# Autodesk Inventor assembly: Intake V3
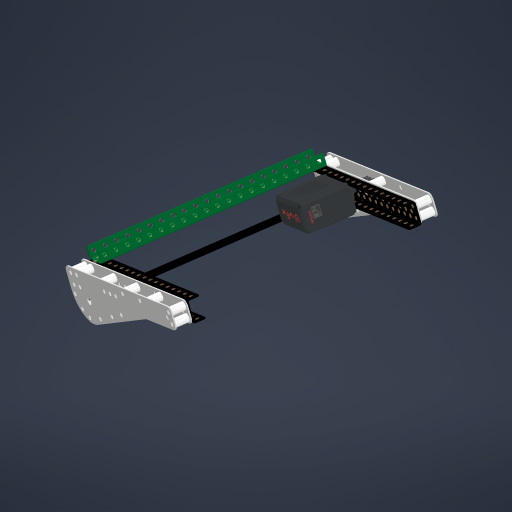
[picture p0: Inventor's stored thumbnail of the model, 512x512]
Saved by Autodesk Inventor 2023.4 (Build 274418000, 418)
## iProperties
Created: 2023-12-16
Part Number: Intake V3
Document SubType Name: Assembly
Designer: diego
Author: diego
## Documents named in this file (17)
- C:\Users\Meer\OneDrive\Documents\GitHub\2024-599Z\Cad\NEW Intake\plan x intake.iam
- C:\Users\Meer\OneDrive\Documents\GitHub\2024-599Z\Cad\Library\VEX-CAD-Inventor-1.4.0\Structure\C Channel\Aluminum 1x2x1\Alu C 1x2x1x17.ipt
- C:\Users\Meer\OneDrive\Documents\GitHub\2024-599Z\Cad\Library\VEX-CAD-Inventor-1.4.0\Motion\Shaft HS\HS Spacer\HSpacer .0625.ipt
- C:\Users\Meer\OneDrive\Documents\GitHub\2024-599Z\Cad\Library\VEX-CAD-Inventor-1.4.0\Motion\Shaft HS\Shaft HS\Shaft HS 11.0 in.ipt
- C:\Users\Meer\OneDrive\Documents\GitHub\2024-599Z\Cad\Library\VEX-CAD-Inventor-1.4.0\Motion\Sprockets\6P Sprocket\6P 8T Sprocket, No Insert.iam
- C:\Users\Meer\OneDrive\Documents\GitHub\2024-599Z\Cad\Library\VEX-CAD-Inventor-1.4.0\Motion\Shaft HS\Low Profile HS Shaft Collar.ipt
- C:\Users\Meer\OneDrive\Documents\GitHub\2024-599Z\Cad\Library\VEX-CAD-Inventor-1.4.0\Motion\Spacers\Spacer Nylon .313 OD\NSpacer .313 OD x .500.ipt
- C:\Users\Meer\OneDrive\Documents\GitHub\2024-599Z\Cad\Library\VEX-CAD-Inventor-1.4.0\Motion\Spacers\Spacer Nylon .313 OD.ipt
- C:\Users\Meer\OneDrive\Documents\GitHub\2024-599Z\Cad\Library\VEX-CAD-Inventor-1.4.0\Motion\Spacers\Spacer Nylon .313 OD\NSpacer .313 OD x .125.ipt
- C:\Users\Meer\OneDrive\Documents\GitHub\2024-599Z\Cad\Library\VEX-CAD-Inventor-1.4.0\Motion\Sprockets\6P Sprocket.iam
- C:\Users\Meer\OneDrive\Documents\GitHub\2024-599Z\Cad\Library\VEX-CAD-Inventor-1.4.0\Motion\Shaft HS\HS Spacer.ipt
- C:\Users\Meer\OneDrive\Documents\GitHub\2024-599Z\Cad\Library\VEX-CAD-Inventor-1.4.0\Motion\Sprockets\6P Sprocket\6P 8T Sprocket, Square.iam
- C:\Users\Meer\OneDrive\Documents\GitHub\2024-599Z\Cad\Library\VEX-CAD-Inventor-1.4.0\Structure\C Channel\Aluminum 1x2x1\Alu C 1x2x1x20.ipt
- C:\Users\Meer\OneDrive\Documents\GitHub\2024-599Z\Cad\Library\VEX-CAD-Inventor-1.4.0\Motion\Shaft HS\Shaft HS.ipt
- C:\Users\Meer\OneDrive\Documents\GitHub\2024-599Z\Cad\NEW CNC Poly\intake poly x.ipt
- C:\Users\Meer\OneDrive\Documents\GitHub\2024-599Z\Cad\Library\VEX-CAD-Inventor-1.4.0\Electronics\Motors with Screws\SteelM-StarS.iam
- C:\Users\Meer\OneDrive\Documents\GitHub\2024-599Z\Cad\Library\VEX-CAD-Inventor-1.4.0\Electronics\Motors with Screws.iam
## Components (78 placed, 11 different names)
1. Shaft HS 11.0 in:1
2. Alu C 1x2x1x17:1 — Insert:138, Insert:139, Insert:146, Insert:147, Insert:208, Insert:209
3. Alu C 1x2x1x17:2 — Insert:136, Insert:137, Insert:205, Insert:206
4. 6P 8T Sprocket, No Insert:4 [sub-assembly] — Insert:24, Insert:39
5. HSpacer .0625:8 — Insert:24
6. HSpacer .0625:12 — Insert:39
7. NSpacer .313 OD x .500:1 — Insert:71, Insert:160
8. NSpacer .313 OD x .500:2 — Insert:65, Insert:161
9. NSpacer .313 OD x .500:4 — Insert:72, Insert:159
10. NSpacer .313 OD x .500:6 — Insert:63, Insert:150
11. NSpacer .313 OD x .500:8 — Insert:74, Insert:157
12. NSpacer .313 OD x .500:9 — Insert:62
13. NSpacer .313 OD x .500:10 — Insert:61
14. NSpacer .313 OD x .500:12 — Insert:67, Insert:154
15. NSpacer .313 OD x .500:13 — Insert:73, Insert:158
16. NSpacer .313 OD x .500:15 — Insert:69, Insert:156
17. NSpacer .313 OD x .125:19 — Insert:61
18. NSpacer .313 OD x .125:20 — Insert:63
19. NSpacer .313 OD x .125:21 — Insert:65
20. NSpacer .313 OD x .125:23 — Insert:62, Insert:201
21. NSpacer .313 OD x .125:24 — Insert:67
22. NSpacer .313 OD x .125:26 — Insert:69, Insert:200
23. NSpacer .313 OD x .125:27 — Insert:71
24. NSpacer .313 OD x .125:29 — Insert:72
25. NSpacer .313 OD x .125:30 — Insert:73
26. NSpacer .313 OD x .125:31 — Insert:74
27. NSpacer .313 OD x .500:34 — Insert:163
28. NSpacer .313 OD x .500:35 — Insert:162
29. NSpacer .313 OD x .500:37 — Insert:153
30. NSpacer .313 OD x .125:47
31. NSpacer .313 OD x .125:50
32. NSpacer .313 OD x .125:59
33. Low Profile HS Shaft Collar:4
34. HSpacer .0625:14 — Insert:135
35. HSpacer .0625:15 — Insert:134, Insert:210
36. 6P 8T Sprocket, Square:6 [sub-assembly] — Insert:134, Insert:135
37. Alu C 1x2x1x20:1 — Insert:136, Insert:137, Insert:138, Insert:139
38. intake poly x:1 — Insert:146, Insert:147, Insert:150, Insert:153, Insert:154, Insert:156, Insert:157, Insert:158, Insert:159, Insert:160, Insert:161, Insert:162, Insert:163, Insert:210
39. intake poly x:2 — Insert:202, Insert:203, Insert:204, Insert:205, Insert:206
40. NSpacer .313 OD x .500:65
41. NSpacer .313 OD x .500:66
42. NSpacer .313 OD x .500:67
43. NSpacer .313 OD x .500:68
44. NSpacer .313 OD x .500:69
45. NSpacer .313 OD x .500:70
46. NSpacer .313 OD x .500:71
47. NSpacer .313 OD x .500:72
48. NSpacer .313 OD x .500:73 — Insert:198
49. NSpacer .313 OD x .500:74 — Insert:199
50. NSpacer .313 OD x .500:75
51. NSpacer .313 OD x .500:76
52. NSpacer .313 OD x .500:77
53. NSpacer .313 OD x .500:78
54. NSpacer .313 OD x .500:79
55. NSpacer .313 OD x .125:80
56. NSpacer .313 OD x .125:81
57. NSpacer .313 OD x .125:82 — Insert:203
58. NSpacer .313 OD x .125:83
59. NSpacer .313 OD x .125:84
60. NSpacer .313 OD x .125:85
61. NSpacer .313 OD x .125:86 — Insert:204
62. NSpacer .313 OD x .125:87
63. NSpacer .313 OD x .125:88
64. NSpacer .313 OD x .125:89 — Insert:202
65. NSpacer .313 OD x .125:90
66. NSpacer .313 OD x .125:91
67. NSpacer .313 OD x .125:92
68. NSpacer .313 OD x .125:93
69. NSpacer .313 OD x .125:94
70. NSpacer .313 OD x .500:95
71. NSpacer .313 OD x .500:96
72. NSpacer .313 OD x .500:97
73. NSpacer .313 OD x .125:98
74. NSpacer .313 OD x .125:99
75. NSpacer .313 OD x .125:100
76. intake poly x:3 — Insert:198, Insert:199
77. intake poly x:4 — Insert:200, Insert:201
78. SteelM-StarS:1 [sub-assembly] — Insert:208, Insert:209
## Relationships (80: Insert 80)
- Insert:24: 6P 8T Sprocket, No Insert:4 ↔ HSpacer .0625:8
- Insert:39: 6P 8T Sprocket, No Insert:4 ↔ HSpacer .0625:12
- Insert:61: NSpacer .313 OD x .500:10 ↔ NSpacer .313 OD x .125:19
- Insert:62: NSpacer .313 OD x .500:9 ↔ NSpacer .313 OD x .125:23
- Insert:63: NSpacer .313 OD x .500:6 ↔ NSpacer .313 OD x .125:20
- Insert:65: NSpacer .313 OD x .500:2 ↔ NSpacer .313 OD x .125:21
- Insert:67: NSpacer .313 OD x .500:12 ↔ NSpacer .313 OD x .125:24
- Insert:69: NSpacer .313 OD x .500:15 ↔ NSpacer .313 OD x .125:26
- Insert:71: NSpacer .313 OD x .500:1 ↔ NSpacer .313 OD x .125:27
- Insert:72: NSpacer .313 OD x .500:4 ↔ NSpacer .313 OD x .125:29
- Insert:73: NSpacer .313 OD x .500:13 ↔ NSpacer .313 OD x .125:30
- Insert:74: NSpacer .313 OD x .500:8 ↔ NSpacer .313 OD x .125:31
- [Insert]: NSpacer .313 OD x .500:34 ↔ NSpacer .313 OD x .125:47
- [Insert]: NSpacer .313 OD x .500:37 ↔ NSpacer .313 OD x .125:50
- [Insert]: NSpacer .313 OD x .500:35 ↔ NSpacer .313 OD x .125:59
- Insert:134: HSpacer .0625:15 ↔ 6P 8T Sprocket, Square:6
- Insert:135: HSpacer .0625:14 ↔ 6P 8T Sprocket, Square:6
- Insert:136: Alu C 1x2x1x17:2 ↔ Alu C 1x2x1x20:1
- Insert:137: Alu C 1x2x1x17:2 ↔ Alu C 1x2x1x20:1
- Insert:138: Alu C 1x2x1x17:1 ↔ Alu C 1x2x1x20:1
- Insert:139: Alu C 1x2x1x17:1 ↔ Alu C 1x2x1x20:1
- Insert:146: Alu C 1x2x1x17:1 ↔ intake poly x:1
- Insert:147: Alu C 1x2x1x17:1 ↔ intake poly x:1
- Insert:150: NSpacer .313 OD x .500:6 ↔ intake poly x:1
- Insert:153: NSpacer .313 OD x .500:37 ↔ intake poly x:1
- Insert:154: NSpacer .313 OD x .500:12 ↔ intake poly x:1
- Insert:156: NSpacer .313 OD x .500:15 ↔ intake poly x:1
- Insert:157: NSpacer .313 OD x .500:8 ↔ intake poly x:1
- Insert:158: NSpacer .313 OD x .500:13 ↔ intake poly x:1
- Insert:159: NSpacer .313 OD x .500:4 ↔ intake poly x:1
- Insert:160: NSpacer .313 OD x .500:1 ↔ intake poly x:1
- Insert:161: NSpacer .313 OD x .500:2 ↔ intake poly x:1
- Insert:162: NSpacer .313 OD x .500:35 ↔ intake poly x:1
- Insert:163: NSpacer .313 OD x .500:34 ↔ intake poly x:1
- [Insert]: NSpacer .313 OD x .500:67 ↔ NSpacer .313 OD x .125:80
- [Insert]: NSpacer .313 OD x .500:71 ↔ NSpacer .313 OD x .125:81
- [Insert]: NSpacer .313 OD x .500:74 ↔ NSpacer .313 OD x .125:82
- [Insert]: NSpacer .313 OD x .500:73 ↔ NSpacer .313 OD x .125:86
- [Insert]: NSpacer .313 OD x .500:70 ↔ NSpacer .313 OD x .125:83
- [Insert]: NSpacer .313 OD x .500:75 ↔ NSpacer .313 OD x .125:85
- [Insert]: NSpacer .313 OD x .500:66 ↔ NSpacer .313 OD x .125:84
- [Insert]: NSpacer .313 OD x .500:69 ↔ NSpacer .313 OD x .125:88
- [Insert]: NSpacer .313 OD x .500:76 ↔ NSpacer .313 OD x .125:87
- [Insert]: NSpacer .313 OD x .500:78 ↔ NSpacer .313 OD x .125:91
- [Insert]: NSpacer .313 OD x .500:79 ↔ NSpacer .313 OD x .125:89
- [Insert]: NSpacer .313 OD x .500:65 ↔ NSpacer .313 OD x .125:90
- [Insert]: NSpacer .313 OD x .500:68 ↔ NSpacer .313 OD x .125:92
- [Insert]: NSpacer .313 OD x .500:77 ↔ NSpacer .313 OD x .125:93
- [Insert]: NSpacer .313 OD x .500:72 ↔ NSpacer .313 OD x .125:94
- [Insert]: NSpacer .313 OD x .500:95 ↔ NSpacer .313 OD x .125:98
- [Insert]: NSpacer .313 OD x .500:97 ↔ NSpacer .313 OD x .125:99
- [Insert]: NSpacer .313 OD x .500:96 ↔ NSpacer .313 OD x .125:100
- [Insert]: NSpacer .313 OD x .500:71 ↔ intake poly x:3
- [Insert]: NSpacer .313 OD x .500:67 ↔ intake poly x:3
- [Insert]: NSpacer .313 OD x .500:70 ↔ intake poly x:3
- [Insert]: NSpacer .313 OD x .500:75 ↔ intake poly x:3
- [Insert]: NSpacer .313 OD x .500:69 ↔ intake poly x:3
- [Insert]: NSpacer .313 OD x .500:97 ↔ intake poly x:3
- [Insert]: NSpacer .313 OD x .500:76 ↔ intake poly x:3
- [Insert]: NSpacer .313 OD x .500:78 ↔ intake poly x:3
- [Insert]: NSpacer .313 OD x .500:79 ↔ intake poly x:3
- [Insert]: NSpacer .313 OD x .500:72 ↔ intake poly x:3
- [Insert]: NSpacer .313 OD x .500:77 ↔ intake poly x:3
- [Insert]: NSpacer .313 OD x .500:68 ↔ intake poly x:3
- [Insert]: NSpacer .313 OD x .500:65 ↔ intake poly x:3
- [Insert]: NSpacer .313 OD x .500:66 ↔ intake poly x:3
- [Insert]: NSpacer .313 OD x .500:96 ↔ intake poly x:3
- [Insert]: NSpacer .313 OD x .500:95 ↔ intake poly x:3
- Insert:198: NSpacer .313 OD x .500:73 ↔ intake poly x:3
- Insert:199: NSpacer .313 OD x .500:74 ↔ intake poly x:3
- Insert:200: NSpacer .313 OD x .125:26 ↔ intake poly x:4
- Insert:201: NSpacer .313 OD x .125:23 ↔ intake poly x:4
- Insert:202: intake poly x:2 ↔ NSpacer .313 OD x .125:89
- Insert:203: intake poly x:2 ↔ NSpacer .313 OD x .125:82
- Insert:204: intake poly x:2 ↔ NSpacer .313 OD x .125:86
- Insert:205: Alu C 1x2x1x17:2 ↔ intake poly x:2
- Insert:206: Alu C 1x2x1x17:2 ↔ intake poly x:2
- Insert:208: Alu C 1x2x1x17:1 ↔ SteelM-StarS:1
- Insert:209: Alu C 1x2x1x17:1 ↔ SteelM-StarS:1
- Insert:210: HSpacer .0625:15 ↔ intake poly x:1
## Named parameters: d129_d111 = 0 mm, d133_d115 = 0 mm, d141_d124 = 0 mm, d230_d214 = 0 mm, d231_d215 = 0 mm, d232_d216 = 0 mm, d233_d217 = 0 mm, d234_d218 = 0 mm, d235_d219 = 0 mm, d236_d220 = 0 mm, d237_d221 = 0 mm, d238_d222 = 0 mm, d239_d223 = 0 mm, d240_d224 = 0 mm, d241_d225 = 0 mm, d242_d226 = 0 mm, d243_d227 = 0 mm, d244_d228 = 0 mm, d245_d229 = 0 mm, d246_d113 = 0 mm, d247_d114 = 0 mm, d248_d115 = 0 mm, d249_d116 = 0 mm, d250_d117 = 0 mm, d251_d118 = 0 mm, d252_d119 = 0 mm, d253_d120 = 0 mm, d254_d121 = 0 mm, d255_d123 = 0 mm, d256_d124 = 0 mm, d257_d125 = 0 mm, d258_d126 = 0 mm, d259_d129_d111 = 0 mm, d260_d133_d115 = 0 mm, d261_d141_d124 = 0 mm, d262_d111 = 0 mm, d263_d112 = 0 mm
